# Autodesk Inventor assembly: PanelJigAssembly
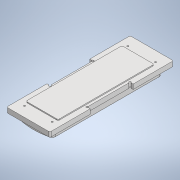
[picture p0: Inventor's stored thumbnail of the model, 180x180]
Saved by Autodesk Inventor 2021 (Build 250183000, 183)
## iProperties
Created: 2020-07-25
Part Number: PanelJigAssembly
Document SubType Name: Assembly
Designer: CASE-SMALL2
Author: CASE-SMALL2
## Documents named in this file (3)
- C:\Users\CASE-SMALL2\Google Drive\Unicorn 2020\CAD_V2\Manufacturing\PanelJigAssembly.iam
- C:\Users\CASE-SMALL2\Google Drive\Unicorn 2020\CAD_V2\Manufacturing\PanelJig.ipt
- C:\Users\CASE-SMALL2\Google Drive\Unicorn 2020\CAD_V2\Back_Panel\Panel\1009799_3D.ipt
## Components (3 placed, 2 different names)
1. PanelJig:1 — Rigid:2, Rigid:3
2. 1009799_3D:1 — Rigid:2
3. 1009799_3D:2 — Rigid:3
## Relationships (2: WeldJoint 2)
- Rigid:2 [WeldJoint]: PanelJig:1 ↔ 1009799_3D:1
- Rigid:3 [WeldJoint]: PanelJig:1 ↔ 1009799_3D:2
